# Autodesk Inventor assembly: Y Axis
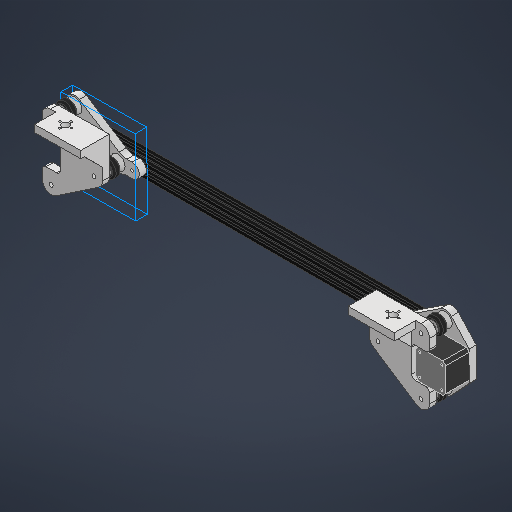
[picture p0: Inventor's stored thumbnail of the model, 512x512]
Saved by Autodesk Inventor 2025.1 (Build 291241000, 241)
## iProperties
Created: 2025-02-05
Part Number: Y Axis
Document SubType Name: Assembly
Designer: jerem
Author: jerem
## Documents named in this file (8)
- C:\Users\jerem\Documents\GitHub\Perovskite-Automated-Synthesis-System\CAD\Gantry\Y Axis.iam
- C:\Users\jerem\Documents\GitHub\Perovskite-Automated-Synthesis-System\CAD\Non 3D Printed Parts\Extrusion\V Extrustion 20x500mm.ipt
- C:\Users\jerem\Documents\GitHub\Perovskite-Automated-Synthesis-System\CAD\Gantry\y axis motor holder.ipt
- C:\Users\jerem\Documents\GitHub\Perovskite-Automated-Synthesis-System\CAD\Gantry\y axis something back.ipt
- C:\Users\jerem\Documents\GitHub\Perovskite-Automated-Synthesis-System\CAD\Gantry\y axis something.ipt
- C:\Users\jerem\Documents\GitHub\Perovskite-Automated-Synthesis-System\CAD\Non 3D Printed Parts\Motors and Servos\NEMA17 Stepper Motor.ipt
- C:\Users\jerem\Documents\GitHub\Perovskite-Automated-Synthesis-System\CAD\Non 3D Printed Parts\Printer Wheel.ipt
- C:\Users\jerem\Documents\GitHub\Perovskite-Automated-Synthesis-System\CAD\Gantry\y axis something_MIR.ipt
## Components (12 placed, 7 different names)
1. V Extrustion 20x500mm:1 — Mate:14, Mate:24, Mate:25
2. y axis motor holder:1 — Mate:1, Mate:2, Mate:4, Mate:5, Mate:6, Mate:7, Mate:8, Mate:9, Mate:10, Mate:11, Mate:13, Mate:14, Mate:25
3. y axis something back:1 — Mate:21, Mate:22, Mate:23, Mate:24
4. y axis something:1 — Mate:4, Mate:5, Mate:12
5. NEMA17 Stepper Motor:1 — Mate:1, Mate:2, Mate:13
6. Printer Wheel:1 — Mate:6, Mate:7
7. Printer Wheel:2 — Mate:8, Mate:11
8. Printer Wheel:3 — Mate:9, Mate:10, Mate:12
9. y axis something_MIR:1 — Mate:15, Mate:16, Mate:17, Mate:18, Mate:19, Mate:20, Mate:21, Mate:22
10. Printer Wheel:4 — Mate:18, Mate:19
11. Printer Wheel:5 — Mate:17, Mate:20, Mate:23
12. Printer Wheel:6 — Mate:15, Mate:16
## Relationships (24: Mate 24)
- Mate:1: y axis motor holder:1 ↔ NEMA17 Stepper Motor:1
- Mate:2: y axis motor holder:1 ↔ NEMA17 Stepper Motor:1
- Mate:4: y axis motor holder:1 ↔ y axis something:1
- Mate:5: y axis motor holder:1 ↔ y axis something:1
- Mate:6: y axis motor holder:1 ↔ Printer Wheel:1
- Mate:7: y axis motor holder:1 ↔ Printer Wheel:1
- Mate:8: y axis motor holder:1 ↔ Printer Wheel:2
- Mate:9: y axis motor holder:1 ↔ Printer Wheel:3
- Mate:10: y axis motor holder:1 ↔ Printer Wheel:3
- Mate:11: y axis motor holder:1 ↔ Printer Wheel:2
- Mate:12: y axis something:1 ↔ Printer Wheel:3
- Mate:13: y axis motor holder:1 ↔ NEMA17 Stepper Motor:1
- Mate:14: V Extrustion 20x500mm:1 ↔ y axis motor holder:1
- Mate:15: y axis something_MIR:1 ↔ Printer Wheel:6
- Mate:16: y axis something_MIR:1 ↔ Printer Wheel:6
- Mate:17: y axis something_MIR:1 ↔ Printer Wheel:5
- Mate:18: y axis something_MIR:1 ↔ Printer Wheel:4
- Mate:19: y axis something_MIR:1 ↔ Printer Wheel:4
- Mate:20: y axis something_MIR:1 ↔ Printer Wheel:5
- Mate:21: y axis something back:1 ↔ y axis something_MIR:1
- Mate:22: y axis something back:1 ↔ y axis something_MIR:1
- Mate:23: y axis something back:1 ↔ Printer Wheel:5
- Mate:24: V Extrustion 20x500mm:1 ↔ y axis something back:1
- Mate:25: V Extrustion 20x500mm:1 ↔ y axis motor holder:1
